# Autodesk Inventor assembly: Cheng Shin C-166-1
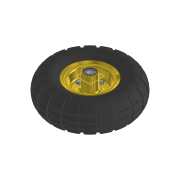
[picture p0: Inventor's stored thumbnail of the model, 180x180]
Saved by Autodesk Inventor 2020.3 (Build 243373000, 373)
## iProperties
Created: 2022-03-26
Part Number: Cheng Shin C-166-1
Document SubType Name: Assembly
Designer: Suriyan.S
Author: Suriyan.S
## Documents named in this file (5)
- D:\T-ROVER_NEW\CAD\Updates\Wheel Attachment\Cheng Shin C-166-1.iam
- D:\T-ROVER_NEW\CAD\Updates\Wheel Attachment\10inchWheel.ipt
- C:\Users\Admin\Documents\Inventor\Content Center Files\R2020\en-US\ISO 8676(2)\ISO 8676 - M8 x 1 x 16 - ISO.ipt
- C:\Users\Admin\Documents\Inventor\Content Center Files\R2020\en-US\ISO 4161\ISO 4161 - M8(1).ipt
- D:\T-ROVER_NEW\CAD\Updates\Wheel Attachment\SKF_6202-2Z.ipt
## Components (11 placed, 4 different names)
1. 10inchWheel:1 — Insert:1, Insert:2, Insert:3, Insert:4, Insert:5, Insert:6, Insert:7, Insert:8, Mate:1, Mate:2, Mate:3, Mate:4
2. SKF_6202-2Z:2 — Mate:1, Mate:2
3. SKF_6202-2Z:1 — Mate:3, Mate:4
4. ISO 8676 M8 x 1 x 16:1 — Insert:1
5. ISO 8676 M8 x 1 x 16:2 — Insert:2
6. ISO 8676 M8 x 1 x 16:3 — Insert:3
7. ISO 8676 M8 x 1 x 16:4 — Insert:4
8. ISO 4161 M8:1 — Insert:5
9. ISO 4161 M8:2 — Insert:6
10. ISO 4161 M8:3 — Insert:7
11. ISO 4161 M8:4 — Insert:8
## Relationships (12: Insert 8, Mate 4)
- Insert:1: 10inchWheel:1 ↔ ISO 8676 M8 x 1 x 16:1
- Insert:2: 10inchWheel:1 ↔ ISO 8676 M8 x 1 x 16:2
- Insert:3: 10inchWheel:1 ↔ ISO 8676 M8 x 1 x 16:3
- Insert:4: 10inchWheel:1 ↔ ISO 8676 M8 x 1 x 16:4
- Insert:5: 10inchWheel:1 ↔ ISO 4161 M8:1
- Insert:6: 10inchWheel:1 ↔ ISO 4161 M8:2
- Insert:7: 10inchWheel:1 ↔ ISO 4161 M8:3
- Insert:8: 10inchWheel:1 ↔ ISO 4161 M8:4
- Mate:1: 10inchWheel:1 ↔ SKF_6202-2Z:2
- Mate:2: 10inchWheel:1 ↔ SKF_6202-2Z:2
- Mate:3: 10inchWheel:1 ↔ SKF_6202-2Z:1
- Mate:4: 10inchWheel:1 ↔ SKF_6202-2Z:1
